# Autodesk Inventor assembly: Flywheel Assembly
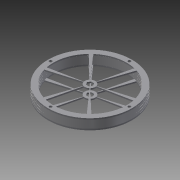
[picture p0: Inventor's stored thumbnail of the model, 180x180]
Saved by Autodesk Inventor 2013 (Build 170138000, 138)
## iProperties
Created: 2013-01-17
Part Number: Flywheel Assembly
Document SubType Name: Assembly
Designer: actoennies
Mass: 1217.46 g
Surface Area: 1466.84 cm^2
Volume: 244.354 cm^3
Density: 4.98237 g/cm^3
Author: actoennies
## Documents named in this file (3)
- \\NNHSSRV2.hs.sd203.org\ACToennies$\frc2013CAD-master\Launcher\Shooter\Flywheel Assembly.iam
- \\NNHSSRV2.hs.sd203.org\ACToennies$\frc2013CAD-master\Launcher\Shooter\Flywheel Hub.ipt
- \\NNHSSRV2.hs.sd203.org\ACToennies$\frc2013CAD-master\Launcher\Shooter\Flywheel Spacer.ipt
## Components (5 placed, 2 different names)
1. Flywheel Hub:1 — Insert:1, Insert:2
2. Flywheel Hub:2 — Insert:7, Insert:8
3. Flywheel Spacer:1 — Insert:5, Insert:6, Insert:7, Insert:8
4. Flywheel Spacer:2 — Insert:3, Insert:4, Insert:5, Insert:6
5. Flywheel Spacer:3 — Insert:1, Insert:2, Insert:3, Insert:4
## Relationships (8: Insert 8)
- Insert:1: Flywheel Hub:1 ↔ Flywheel Spacer:3
- Insert:2: Flywheel Hub:1 ↔ Flywheel Spacer:3
- Insert:3: Flywheel Spacer:2 ↔ Flywheel Spacer:3
- Insert:4: Flywheel Spacer:2 ↔ Flywheel Spacer:3
- Insert:5: Flywheel Spacer:1 ↔ Flywheel Spacer:2
- Insert:6: Flywheel Spacer:1 ↔ Flywheel Spacer:2
- Insert:7: Flywheel Hub:2 ↔ Flywheel Spacer:1
- Insert:8: Flywheel Hub:2 ↔ Flywheel Spacer:1
